# Autodesk Inventor assembly: CMV12000 Extraction Tool V01
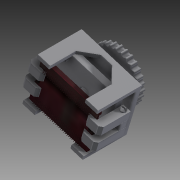
[picture p0: Inventor's stored thumbnail of the model, 180x180]
Saved by Autodesk Inventor 2015 (Build 190159000, 159)
## iProperties
Created: 2016-09-16
Part Number: CMV12000 Extraction Tool V01
Document SubType Name: Assembly
Designer: spichelh
Author: spichelh
## Documents named in this file (6)
- C:\Users\spichelh\Documents\GitHub\beta-hardware\Manufacturing Tools\CMV12000 Extraction Tool V01\CMV12000 Extraction Tool V01.iam
- C:\Users\spichelh\Documents\GitHub\beta-hardware\Manufacturing Tools\CMV12000 Extraction Tool V01\CMV12000v1.ipt
- C:\Users\spichelh\Documents\GitHub\beta-hardware\Manufacturing Tools\CMV12000 Extraction Tool V01\arms01.ipt
- C:\Users\spichelh\Documents\GitHub\beta-hardware\Manufacturing Tools\CMV12000 Extraction Tool V01\base.ipt
- C:\Users\spichelh\Documents\GitHub\beta-hardware\Manufacturing Tools\CMV12000 Extraction Tool V01\mover01.ipt
- C:\Users\spichelh\Documents\GitHub\beta-hardware\Manufacturing Tools\CMV12000 Extraction Tool V01\Knob01.ipt
## Components (6 placed, 5 different names)
1. CMV12000v1:1 — Mate:3, Flush:8, Flush:9, Mate:7, Mate:11, Mate:14
2. arms01:1 — Rotational:2, Mate:14
3. arms01:2 — Rotational:1, Mate:11
4. base:1 — Flush:8, Flush:9, Mate:7, Mate:8, Mate:9, Mate:10, Mate:12
5. mover01:1 — Mate:8, Mate:9, Rotational:1, Mate:10, Mate:13, Rotational:2
6. Knob01:1 — Mate:12, Mate:13
## Relationships (13: Mate 9, Flush 2, RevoluteJoint 2)
- Mate:3: CMV12000v1:1
- Flush:8 (-3 mm): CMV12000v1:1 ↔ base:1
- Flush:9 (-1 mm): CMV12000v1:1 ↔ base:1
- Mate:7 (1 mm): CMV12000v1:1 ↔ base:1
- Mate:8: base:1 ↔ mover01:1
- Mate:9: base:1 ↔ mover01:1
- Rotational:1 [RevoluteJoint]: arms01:2 ↔ mover01:1
- Mate:10 (7 mm): base:1 ↔ mover01:1
- Mate:11: CMV12000v1:1 ↔ arms01:2
- Mate:12: base:1 ↔ Knob01:1
- Mate:13: mover01:1 ↔ Knob01:1
- Rotational:2 [RevoluteJoint]: arms01:1 ↔ mover01:1
- Mate:14: CMV12000v1:1 ↔ arms01:1
